# Autodesk Inventor assembly: 1 Piece Support Assembly
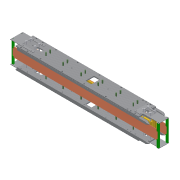
[picture p0: Inventor's stored thumbnail of the model, 180x180]
Saved by Autodesk Inventor 2011 (Build 150239000, 239)
## iProperties
Created: 2006-06-01
Part Number: 1 Piece Support Assembly
Document SubType Name: Assembly
Designer: Jon
Author: Jon
## Documents named in this file (8)
- C:\Users\Joe\Inventor\EDM\Field Plates\1 Piece Support Assembly.iam
- C:\Users\Joe\Inventor\EDM\Field Plates\1 Piece Support Plate.ipt
- C:\Users\Joe\Inventor\EDM\Field Plates\Original Field Plates\Long rod.ipt
- C:\Users\Joe\Inventor\EDM\Field Plates\Field Plate & Rods.iam
- C:\Users\Joe\Inventor\EDM\Field Plates\top support extension.ipt
- C:\Users\Joe\Inventor\EDM\Field Plates\bottom support extension.ipt
- C:\Users\Joe\Inventor\EDM\Field Plates\feet.ipt
- C:\Users\Joe\Inventor\EDM\Field Plates\rf transmission plate.ipt
## Components (18 placed, 7 different names)
1. 1 Piece Support Plate:1 — Mate:1, Mate:2, Mate:3, Mate:4, Insert:1, Insert:4, Mate:41, Mate:42, Mate:43, Mate:55, Mate:56, Mate:57
2. Field Plate & Rods:1 [sub-assembly] — Mate:3, Mate:4, Mate:5, Mate:6, Flush:1
3. Field Plate & Rods:2 [sub-assembly] — Mate:1, Mate:2, Flush:2
4. 1 Piece Support Plate:2 — Mate:5, Mate:6, Flush:1, Flush:2, Insert:2, Insert:3, Mate:44, Mate:45, Mate:46, Mate:52, Mate:53, Mate:54
5. Long rod:1 — Insert:1
6. Long rod:2 — Insert:2
7. Long rod:3 — Insert:3
8. Long rod:4 — Insert:4
9. top support extension:1 — Mate:41, Mate:42, Mate:43, Mate:62, Mate:63, Mate:64
10. top support extension:2 — Mate:44, Mate:45, Mate:46, Mate:50, Mate:61
11. bottom support extension:1 — Mate:55, Mate:56, Mate:57, Mate:65, Mate:66
12. feet:1 — Mate:15, Mate:16, Mate:17, Mate:50, Mate:62, Mate:64
13. feet:2 — Mate:24, Mate:30, Mate:47, Mate:61, Mate:63
14. feet:3 — Mate:20, Mate:40, Mate:66
15. feet:4 — Mate:21, Mate:22, Mate:23, Mate:65
16. rf transmission plate:1 — Mate:15, Mate:16, Mate:17, Mate:20, Mate:40
17. rf transmission plate:2 — Mate:21, Mate:22, Mate:23, Mate:24, Mate:30, Mate:47
18. bottom support extension:2 — Mate:52, Mate:53, Mate:54
## Relationships (42: Mate 36, Insert 4, Flush 2)
- Mate:1: 1 Piece Support Plate:1 ↔ Field Plate & Rods:2
- Mate:2: 1 Piece Support Plate:1 ↔ Field Plate & Rods:2
- Mate:3: 1 Piece Support Plate:1 ↔ Field Plate & Rods:1
- Mate:4: 1 Piece Support Plate:1 ↔ Field Plate & Rods:1
- Mate:5: Field Plate & Rods:1 ↔ 1 Piece Support Plate:2
- Mate:6: Field Plate & Rods:1 ↔ 1 Piece Support Plate:2
- Flush:1 (-10 mm): Field Plate & Rods:1 ↔ 1 Piece Support Plate:2
- Flush:2 (-10 mm): Field Plate & Rods:2 ↔ 1 Piece Support Plate:2
- Insert:1: 1 Piece Support Plate:1 ↔ Long rod:1
- Insert:2: 1 Piece Support Plate:2 ↔ Long rod:2
- Insert:3: 1 Piece Support Plate:2 ↔ Long rod:3
- Insert:4: 1 Piece Support Plate:1 ↔ Long rod:4
- Mate:15: feet:1 ↔ rf transmission plate:1
- Mate:16: feet:1 ↔ rf transmission plate:1
- Mate:17: feet:1 ↔ rf transmission plate:1
- Mate:20: feet:3 ↔ rf transmission plate:1
- Mate:21: feet:4 ↔ rf transmission plate:2
- Mate:22: feet:4 ↔ rf transmission plate:2
- Mate:23: feet:4 ↔ rf transmission plate:2
- Mate:24: feet:2 ↔ rf transmission plate:2
- Mate:30: feet:2 ↔ rf transmission plate:2
- Mate:40: feet:3 ↔ rf transmission plate:1
- Mate:41: 1 Piece Support Plate:1 ↔ top support extension:1
- Mate:42: 1 Piece Support Plate:1 ↔ top support extension:1
- Mate:43: 1 Piece Support Plate:1 ↔ top support extension:1
- Mate:44: 1 Piece Support Plate:2 ↔ top support extension:2
- Mate:45: 1 Piece Support Plate:2 ↔ top support extension:2
- Mate:46: 1 Piece Support Plate:2 ↔ top support extension:2
- Mate:47: feet:2 ↔ rf transmission plate:2
- Mate:50: top support extension:2 ↔ feet:1
- Mate:52: 1 Piece Support Plate:2 ↔ bottom support extension:2
- Mate:53: 1 Piece Support Plate:2 ↔ bottom support extension:2
- Mate:54: 1 Piece Support Plate:2 ↔ bottom support extension:2
- Mate:55: 1 Piece Support Plate:1 ↔ bottom support extension:1
- Mate:56: 1 Piece Support Plate:1 ↔ bottom support extension:1
- Mate:57: 1 Piece Support Plate:1 ↔ bottom support extension:1
- Mate:61: top support extension:2 ↔ feet:2
- Mate:62: top support extension:1 ↔ feet:1
- Mate:63: top support extension:1 ↔ feet:2
- Mate:64: top support extension:1 ↔ feet:1
- Mate:65: bottom support extension:1 ↔ feet:4
- Mate:66: bottom support extension:1 ↔ feet:3
